# Autodesk Inventor assembly: YAxis_Carriage
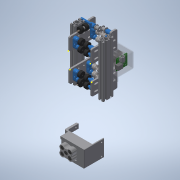
[picture p0: Inventor's stored thumbnail of the model, 180x180]
Saved by Autodesk Inventor 2021 (Build 250183000, 183)
## iProperties
Created: 2021-02-02
Part Number: YAxis_Carriage
Document SubType Name: Assembly
Designer: Jorian Brusind
Author: Jorian Brusind
## Documents named in this file (16)
- C:\Users\Jorian Brusind\Documents\GitHub\PersonalProjects\HyperRail\Inventor Files\YAxis_Carriage.iam
- C:\Users\Jorian Brusind\Documents\GitHub\PersonalProjects\Inventor Projects\Useful models\NEMA_Steppers\nema-17-stepper-motor-with-v2-damper-1.snapshot.3\Nema 17  Stepper Motor length 34mm.ipt
- C:\Users\Jorian Brusind\Documents\GitHub\PersonalProjects\HyperRail\Inventor Files\SmallBelt_Pulley.ipt
- C:\Users\Jorian Brusind\Documents\GitHub\PersonalProjects\Inventor Projects\Useful models\Metric bolt\Bolt M3 30mm.ipt
- C:\Users\Jorian Brusind\Documents\GitHub\PersonalProjects\HyperRail\Inventor Files\small_belt_loop.ipt
- C:\Users\Jorian Brusind\Documents\GitHub\PersonalProjects\HyperRail\PCB Files\Integrated Stepper Motor Driver\ExportSTEP\Main.iam
- C:\Users\Jorian Brusind\Documents\GitHub\PersonalProjects\HyperRail\Inventor Files\rededge-micasense-1.snapshot.3\PND_CAM_MSRE.ipt
- C:\Users\Jorian Brusind\Documents\GitHub\PersonalProjects\HyperRail\Inventor Files\Camera_Mount.ipt
- C:\Users\Jorian Brusind\Documents\GitHub\PersonalProjects\HyperRail\Inventor Files\NEMA17_Shroud.ipt
- C:\Users\Jorian Brusind\Documents\GitHub\PersonalProjects\HyperRail\Inventor Files\Buffer.iam
- C:\Users\Jorian Brusind\Documents\GitHub\PersonalProjects\HyperRail\Inventor Files\X_Carriage_V2_0.iam
- C:\Users\Jorian Brusind\Documents\GitHub\PersonalProjects\HyperRail\Inventor Files\X_CarriageR_V2_0.iam
- C:\Users\Jorian Brusind\Documents\GitHub\PersonalProjects\HyperRail\Inventor Files\X_CarriageR_V2_1.iam
- C:\Users\Jorian Brusind\Documents\GitHub\PersonalProjects\HyperRail\Inventor Files\X_Carriage_V2_1.iam
- C:\Users\Jorian Brusind\Documents\GitHub\PersonalProjects\Inventor Projects\Useful models\8020_Sets\IPT_20_Series\IPT_20_Series\20-2040_200mm.ipt
- C:\Users\Jorian Brusind\Documents\GitHub\PersonalProjects\HyperRail\Inventor Files\10mm_Idle_Pulley_3M.ipt
## Components (20 placed, 15 different names)
1. Nema 17  Stepper Motor length 34mm:1 — Mate:13, Mate:14, Mate:36, Mate:42, Flush:14, Flush:15, Angle:1, Mate:171, Mate:172, Mate:173
2. SmallBelt_Pulley:1 — Mate:13, Mate:14, Mate:37, Flush:94
3. small_belt_loop:1 — Mate:36, Mate:37, Angle:1
4. Main:1 [sub-assembly] — Mate:42, Flush:14, Flush:15
5. PND_CAM_MSRE:1 — Mate:47, Mate:48, Mate:49
6. Camera_Mount:1 — Mate:47, Mate:48, Mate:49
7. NEMA17_Shroud:1 — Mate:169, Mate:171, Mate:172, Mate:173, Mate:178, Mate:179, Mate:180, Mate:181, Mate:182, Mate:185
8. 20-2040_200mm:1 — Flush:74, Flush:75, Mate:151, Mate:157, Mate:158, Flush:76, Flush:77, Flush:78, Flush:79, Mate:161, Flush:80, Mate:175, Flush:89
9. 20-2040_200mm:2 — Flush:74, Flush:75, Mate:155, Mate:156, Mate:160, Mate:169, Mate:174
10. X_CarriageR_V2_0:4 [sub-assembly] — Mate:161, Flush:80, Mate:162, Mate:163, Flush:85, Mate:166, Mate:167, Flush:86, Flush:90
11. X_Carriage_V2_1:3 [sub-assembly] — Mate:160, Mate:163, Flush:85, Mate:166, Mate:167, Mate:185
12. Buffer:4 [sub-assembly] — Mate:157, Flush:76, Flush:77, Mate:162
13. Buffer:5 [sub-assembly] — Mate:158, Flush:78, Flush:79
14. Bolt M3 30mm:2 — Mate:183, Mate:184
15. X_Carriage_V2_0:1 [sub-assembly] — Mate:175, Flush:86, Flush:87, Flush:88, Flush:89, Mate:176, Flush:90, Mate:177
16. X_CarriageR_V2_1:1 [sub-assembly] — Mate:174, Flush:87, Flush:88, Mate:176, Mate:177, Mate:182
17. 10mm_Idle_Pulley_3M:1 — Mate:180, Flush:93
18. 10mm_Idle_Pulley_3M:2 — Mate:179, Flush:91
19. 10mm_Idle_Pulley_3M:3 — Mate:181, Flush:92
20. 10mm_Idle_Pulley_3M:4 — Mate:178, Flush:91, Flush:92, Flush:93, Flush:94, Mate:183, Mate:184
## Relationships (55: Mate 35, Flush 19, Angle 1)
- Mate:13: Nema 17  Stepper Motor length 34mm:1 ↔ SmallBelt_Pulley:1
- Mate:14: Nema 17  Stepper Motor length 34mm:1 ↔ SmallBelt_Pulley:1
- Mate:36: Nema 17  Stepper Motor length 34mm:1 ↔ small_belt_loop:1
- Mate:37 (2 mm): SmallBelt_Pulley:1 ↔ small_belt_loop:1
- Mate:42 (5 mm): Nema 17  Stepper Motor length 34mm:1 ↔ Main:1
- Flush:14: Nema 17  Stepper Motor length 34mm:1 ↔ Main:1
- Flush:15: Nema 17  Stepper Motor length 34mm:1 ↔ Main:1
- Mate:47: PND_CAM_MSRE:1 ↔ Camera_Mount:1
- Mate:48: PND_CAM_MSRE:1 ↔ Camera_Mount:1
- Mate:49: PND_CAM_MSRE:1 ↔ Camera_Mount:1
- Flush:74: 20-2040_200mm:1 ↔ 20-2040_200mm:2
- Flush:75: 20-2040_200mm:1 ↔ 20-2040_200mm:2
- Mate:151: 20-2040_200mm:1
- Mate:155: 20-2040_200mm:2
- Mate:156: 20-2040_200mm:2
- Mate:157: 20-2040_200mm:1 ↔ Buffer:4
- Mate:158: 20-2040_200mm:1 ↔ Buffer:5
- Flush:76: 20-2040_200mm:1 ↔ Buffer:4
- Flush:77: 20-2040_200mm:1 ↔ Buffer:4
- Flush:78: 20-2040_200mm:1 ↔ Buffer:5
- Flush:79: 20-2040_200mm:1 ↔ Buffer:5
- Mate:160: 20-2040_200mm:2 ↔ X_Carriage_V2_1:3
- Mate:161: 20-2040_200mm:1 ↔ X_CarriageR_V2_0:4
- Flush:80: 20-2040_200mm:1 ↔ X_CarriageR_V2_0:4
- Mate:162 (4 mm): X_CarriageR_V2_0:4 ↔ Buffer:4
- Mate:163: X_CarriageR_V2_0:4 ↔ X_Carriage_V2_1:3
- Flush:85: X_CarriageR_V2_0:4 ↔ X_Carriage_V2_1:3
- Mate:166 (10 mm): X_CarriageR_V2_0:4 ↔ X_Carriage_V2_1:3
- Mate:167: X_CarriageR_V2_0:4 ↔ X_Carriage_V2_1:3
- Mate:169: NEMA17_Shroud:1 ↔ 20-2040_200mm:2
- Angle:1 (0 deg): Nema 17  Stepper Motor length 34mm:1 ↔ small_belt_loop:1
- Mate:171: Nema 17  Stepper Motor length 34mm:1 ↔ NEMA17_Shroud:1
- Mate:172: Nema 17  Stepper Motor length 34mm:1 ↔ NEMA17_Shroud:1
- Mate:173: Nema 17  Stepper Motor length 34mm:1 ↔ NEMA17_Shroud:1
- Mate:174: 20-2040_200mm:2 ↔ X_CarriageR_V2_1:1
- Mate:175: 20-2040_200mm:1 ↔ X_Carriage_V2_0:1
- Flush:86: X_CarriageR_V2_0:4 ↔ X_Carriage_V2_0:1
- Flush:87: X_Carriage_V2_0:1 ↔ X_CarriageR_V2_1:1
- Flush:88: X_Carriage_V2_0:1 ↔ X_CarriageR_V2_1:1
- Flush:89: 20-2040_200mm:1 ↔ X_Carriage_V2_0:1
- Mate:176: X_Carriage_V2_0:1 ↔ X_CarriageR_V2_1:1
- Flush:90: X_CarriageR_V2_0:4 ↔ X_Carriage_V2_0:1
- Mate:177: X_Carriage_V2_0:1 ↔ X_CarriageR_V2_1:1
- Mate:178: NEMA17_Shroud:1 ↔ 10mm_Idle_Pulley_3M:4
- Mate:179: NEMA17_Shroud:1 ↔ 10mm_Idle_Pulley_3M:2
- Mate:180: NEMA17_Shroud:1 ↔ 10mm_Idle_Pulley_3M:1
- Mate:181: NEMA17_Shroud:1 ↔ 10mm_Idle_Pulley_3M:3
- Flush:91: 10mm_Idle_Pulley_3M:2 ↔ 10mm_Idle_Pulley_3M:4
- Flush:92: 10mm_Idle_Pulley_3M:3 ↔ 10mm_Idle_Pulley_3M:4
- Flush:93: 10mm_Idle_Pulley_3M:1 ↔ 10mm_Idle_Pulley_3M:4
- Mate:182: NEMA17_Shroud:1 ↔ X_CarriageR_V2_1:1
- Flush:94: SmallBelt_Pulley:1 ↔ 10mm_Idle_Pulley_3M:4
- Mate:183: Bolt M3 30mm:2 ↔ 10mm_Idle_Pulley_3M:4
- Mate:184: Bolt M3 30mm:2 ↔ 10mm_Idle_Pulley_3M:4
- Mate:185: NEMA17_Shroud:1 ↔ X_Carriage_V2_1:3
